# Autodesk Inventor assembly: Drive2
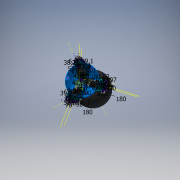
[picture p0: Inventor's stored thumbnail of the model, 180x180]
Saved by Autodesk Inventor 2018.3 (Build 223284000, 284)
## iProperties
Created: 2018-06-30
Part Number: Drive2
Material: Generisch
Document SubType Name: Assembly
Designer: JochenAlt
Author: JochenAlt
## Documents named in this file (4)
- D:\Projects\FlowerPot\CAD\Drive.iam
- D:\Projects\FlowerPot\CAD\Sphere.ipt
- D:\Projects\FlowerPot\CAD\Form.iam
- D:\Projects\FlowerPot\CAD\DriveChain.iam
## Components (5 placed, 3 different names)
1. Sphere:1 — Passend:38, Passend:45, Tangential:1
2. Form:1 [sub-assembly] — Passend:46
3. DriveChain:1 [sub-assembly] — Passend:42, Passend:43, Passend:49, Passend:50, Passend:51, Passend:52
4. DriveChain:2 [sub-assembly] — Passend:41, Passend:42, Passend:44, Tangential:1, Passend:48, Passend:52
5. DriveChain:3 [sub-assembly] — Passend:41, Passend:43, Passend:44, Passend:45, Passend:46, Passend:48, Passend:49, Passend:50, Passend:51
## Relationships (13: Mate 12, Tangent 1)
- Passend:38 [Mate]: Sphere:1
- Passend:41 [Mate]: DriveChain:2 ↔ DriveChain:3
- Passend:42 [Mate]: DriveChain:1 ↔ DriveChain:2
- Passend:43 [Mate]: DriveChain:1 ↔ DriveChain:3
- Passend:44 [Mate]: DriveChain:2 ↔ DriveChain:3
- Passend:45 [Mate]: Sphere:1 ↔ DriveChain:3
- Tangential:1: Sphere:1 ↔ DriveChain:2
- Passend:46 [Mate]: Form:1 ↔ DriveChain:3
- Passend:48 [Mate]: DriveChain:2 ↔ DriveChain:3
- Passend:49 [Mate]: DriveChain:1 ↔ DriveChain:3
- Passend:50 [Mate]: DriveChain:1 ↔ DriveChain:3
- Passend:51 [Mate]: DriveChain:1 ↔ DriveChain:3
- Passend:52 [Mate]: DriveChain:1 ↔ DriveChain:2
